# Autodesk Inventor assembly: BrainBoxV1
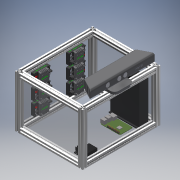
[picture p0: Inventor's stored thumbnail of the model, 180x180]
Saved by Autodesk Inventor 2018 (Build 220112000, 112)
## iProperties
Created: 2019-01-09
Part Number: BrainBoxV1
Document SubType Name: Assembly
Designer: snipe
Author: snipe
## Documents named in this file (14)
- E:\Clark\Assets\BrainBoxV1.iam
- E:\Clark\Assets\Profile_BaseModel_20mm.ipt
- E:\Clark\Assets\Profile_BaseModel_20mm\Profile_BaseModel_20mm-14.ipt
- E:\Clark\Assets\Profile_BaseModel_20mm\Profile_BaseModel_20mm-12.ipt
- E:\Clark\Assets\Profile_BaseModel_20mm\Profile_BaseModel_20mm-11.ipt
- E:\Clark\Assets\PlexiPart\PlexiPart-01.ipt
- E:\Clark\Assets\PlexiPart.ipt
- E:\Clark\Assets\PlexiPart\PlexiPart-02.ipt
- E:\Clark\Assets\PlexiPart\PlexiPart-03.ipt
- E:\Clark\Assets\RPi3Mock.ipt
- E:\Clark\Assets\Netgear Router.ipt
- E:\Clark\Assets\PowerRegulator5V.ipt
- E:\Clark\Assets\Talon.iam
- E:\Clark\Assets\Kinect.iam
## Components (27 placed, 11 different names)
1. Profile_BaseModel_20mm-14:1 — Mate:1, Mate:2, Flush:1, Flush:2, Flush:5, Flush:6, Mate:8, Flush:17, Flush:18, Mate:18, Symmetry:2
2. Profile_BaseModel_20mm-14:2 — Mate:3, Flush:3, Flush:4, Flush:7, Mate:22, Mate:24
3. Profile_BaseModel_20mm-12:5 — Mate:1, Flush:5, Flush:6, Flush:7, Mate:12, Mate:13, Mate:21, Flush:26
4. Profile_BaseModel_20mm-12:6 — Mate:2, Mate:3, Flush:1, Flush:2, Flush:3, Flush:4
5. Profile_BaseModel_20mm-14:7 — Mate:7, Flush:15, Flush:16, Mate:9, Flush:19, Flush:20, Mate:19, Symmetry:2
6. Profile_BaseModel_20mm-14:8 — Mate:10, Flush:21, Flush:22, Mate:11, Flush:23, Flush:24
7. Profile_BaseModel_20mm-12:9 — Mate:20, Mate:27
8. Profile_BaseModel_20mm-12:10 — Mate:50
9. Profile_BaseModel_20mm-11:11 — Mate:7, Flush:15, Flush:16, Mate:8, Flush:17, Flush:18, Mate:48
10. Profile_BaseModel_20mm-11:12 — Mate:9, Flush:19, Flush:20, Mate:14, Mate:17, Mate:26
11. Profile_BaseModel_20mm-11:13 — Mate:10, Flush:21, Flush:22, Mate:51, Mate:55, Flush:37
12. Profile_BaseModel_20mm-11:14 — Mate:11, Flush:23, Flush:24, Mate:23, Mate:25, Mate:54
13. PlexiPart-01:1 — Mate:12, Mate:13, Mate:14, Mate:34, Mate:49, Mate:53
14. PlexiPart-02:3 — Mate:19, Mate:20, Mate:27
15. PlexiPart-02:4 — Mate:21, Mate:22, Flush:26
16. PlexiPart-03:5 — Mate:23, Mate:24, Mate:25
17. PlexiPart-03:6 — Mate:17, Mate:18, Mate:26, Mate:41, Mate:42, Mate:43, Mate:44, Mate:45, Mate:46
18. Talon:7 [sub-assembly] — Mate:41, Flush:28, Flush:31, Mate:47, Symmetry:1
19. Talon:8 [sub-assembly] — Mate:42, Flush:27, Flush:28, Flush:32
20. Talon:9 [sub-assembly] — Mate:43, Flush:27, Flush:33
21. Talon:10 [sub-assembly] — Mate:44, Flush:29, Flush:31, Mate:47, Symmetry:1, Flush:35, Mate:48
22. Talon:11 [sub-assembly] — Mate:45, Flush:29, Flush:30, Flush:32, Flush:35, Flush:36
23. Talon:12 [sub-assembly] — Mate:46, Flush:30, Flush:33, Flush:36
24. RPi3Mock:1 — Mate:34, Mate:52
25. Netgear Router:1 — Mate:49, Mate:50, Mate:51, Mate:52
26. PowerRegulator5V:1 — Mate:53, Mate:54
27. Kinect:1 [sub-assembly] — Mate:55, Flush:37
## Relationships (82: Mate 44, Flush 36, Symmetry 2)
- Mate:1: Profile_BaseModel_20mm-14:1 ↔ Profile_BaseModel_20mm-12:5
- Mate:2: Profile_BaseModel_20mm-14:1 ↔ Profile_BaseModel_20mm-12:6
- Mate:3: Profile_BaseModel_20mm-14:2 ↔ Profile_BaseModel_20mm-12:6
- Flush:1: Profile_BaseModel_20mm-14:1 ↔ Profile_BaseModel_20mm-12:6
- Flush:2: Profile_BaseModel_20mm-14:1 ↔ Profile_BaseModel_20mm-12:6
- Flush:3: Profile_BaseModel_20mm-14:2 ↔ Profile_BaseModel_20mm-12:6
- Flush:4: Profile_BaseModel_20mm-14:2 ↔ Profile_BaseModel_20mm-12:6
- Flush:5: Profile_BaseModel_20mm-14:1 ↔ Profile_BaseModel_20mm-12:5
- Flush:6: Profile_BaseModel_20mm-14:1 ↔ Profile_BaseModel_20mm-12:5
- Flush:7: Profile_BaseModel_20mm-14:2 ↔ Profile_BaseModel_20mm-12:5
- [Mate]: Profile_BaseModel_20mm-14:7 ↔ Profile_BaseModel_20mm-12:9
- [Mate]: Profile_BaseModel_20mm-14:7 ↔ Profile_BaseModel_20mm-12:10
- [Mate]: Profile_BaseModel_20mm-14:8 ↔ Profile_BaseModel_20mm-12:10
- [Flush]: Profile_BaseModel_20mm-14:7 ↔ Profile_BaseModel_20mm-12:10
- [Flush]: Profile_BaseModel_20mm-14:7 ↔ Profile_BaseModel_20mm-12:10
- [Flush]: Profile_BaseModel_20mm-14:8 ↔ Profile_BaseModel_20mm-12:10
- [Flush]: Profile_BaseModel_20mm-14:8 ↔ Profile_BaseModel_20mm-12:10
- [Flush]: Profile_BaseModel_20mm-14:7 ↔ Profile_BaseModel_20mm-12:9
- [Flush]: Profile_BaseModel_20mm-14:7 ↔ Profile_BaseModel_20mm-12:9
- [Flush]: Profile_BaseModel_20mm-14:8 ↔ Profile_BaseModel_20mm-12:9
- Mate:7: Profile_BaseModel_20mm-14:7 ↔ Profile_BaseModel_20mm-11:11
- Flush:15: Profile_BaseModel_20mm-14:7 ↔ Profile_BaseModel_20mm-11:11
- Flush:16: Profile_BaseModel_20mm-14:7 ↔ Profile_BaseModel_20mm-11:11
- Mate:8: Profile_BaseModel_20mm-14:1 ↔ Profile_BaseModel_20mm-11:11
- Flush:17: Profile_BaseModel_20mm-14:1 ↔ Profile_BaseModel_20mm-11:11
- Flush:18: Profile_BaseModel_20mm-14:1 ↔ Profile_BaseModel_20mm-11:11
- Mate:9: Profile_BaseModel_20mm-14:7 ↔ Profile_BaseModel_20mm-11:12
- Flush:19: Profile_BaseModel_20mm-14:7 ↔ Profile_BaseModel_20mm-11:12
- Flush:20: Profile_BaseModel_20mm-14:7 ↔ Profile_BaseModel_20mm-11:12
- Mate:10: Profile_BaseModel_20mm-14:8 ↔ Profile_BaseModel_20mm-11:13
- Flush:21: Profile_BaseModel_20mm-14:8 ↔ Profile_BaseModel_20mm-11:13
- Flush:22: Profile_BaseModel_20mm-14:8 ↔ Profile_BaseModel_20mm-11:13
- Mate:11: Profile_BaseModel_20mm-14:8 ↔ Profile_BaseModel_20mm-11:14
- Flush:23: Profile_BaseModel_20mm-14:8 ↔ Profile_BaseModel_20mm-11:14
- Flush:24: Profile_BaseModel_20mm-14:8 ↔ Profile_BaseModel_20mm-11:14
- Mate:12: Profile_BaseModel_20mm-12:5 ↔ PlexiPart-01:1
- Mate:13: Profile_BaseModel_20mm-12:5 ↔ PlexiPart-01:1
- Mate:14: Profile_BaseModel_20mm-11:12 ↔ PlexiPart-01:1
- Mate:17: Profile_BaseModel_20mm-11:12 ↔ PlexiPart-03:6
- Mate:18: Profile_BaseModel_20mm-14:1 ↔ PlexiPart-03:6
- Mate:19: Profile_BaseModel_20mm-14:7 ↔ PlexiPart-02:3
- Mate:20: Profile_BaseModel_20mm-12:9 ↔ PlexiPart-02:3
- Mate:21: Profile_BaseModel_20mm-12:5 ↔ PlexiPart-02:4
- Mate:22: Profile_BaseModel_20mm-14:2 ↔ PlexiPart-02:4
- Mate:23: Profile_BaseModel_20mm-11:14 ↔ PlexiPart-03:5
- Mate:24: Profile_BaseModel_20mm-14:2 ↔ PlexiPart-03:5
- Flush:26: Profile_BaseModel_20mm-12:5 ↔ PlexiPart-02:4
- Mate:25: Profile_BaseModel_20mm-11:14 ↔ PlexiPart-03:5
- Mate:26: Profile_BaseModel_20mm-11:12 ↔ PlexiPart-03:6
- Mate:27: Profile_BaseModel_20mm-12:9 ↔ PlexiPart-02:3
- Mate:34: PlexiPart-01:1 ↔ RPi3Mock:1
- [Mate]: PlexiPart-03:6 ↔ Talon:10
- [Mate]: PlexiPart-03:6 ↔ Talon:11
- [Mate]: PlexiPart-03:6 ↔ Talon:12
- Mate:41: PlexiPart-03:6 ↔ Talon:7
- Mate:42: PlexiPart-03:6 ↔ Talon:8
- Mate:43: PlexiPart-03:6 ↔ Talon:9
- Flush:27: Talon:8 ↔ Talon:9
- Flush:28: Talon:7 ↔ Talon:8
- Mate:44: PlexiPart-03:6 ↔ Talon:10
- Mate:45: PlexiPart-03:6 ↔ Talon:11
- Mate:46: PlexiPart-03:6 ↔ Talon:12
- Flush:29: Talon:10 ↔ Talon:11
- Flush:30: Talon:11 ↔ Talon:12
- Flush:31: Talon:7 ↔ Talon:10
- Flush:32: Talon:8 ↔ Talon:11
- Flush:33: Talon:9 ↔ Talon:12
- Mate:47 (152.4 mm): Talon:7 ↔ Talon:10
- Symmetry:1: Talon:7 ↔ Talon:10
- Symmetry:2: Profile_BaseModel_20mm-14:1 ↔ Profile_BaseModel_20mm-14:7
- Flush:34
- Flush:35 (57.15 mm): Talon:10 ↔ Talon:11
- Flush:36 (57.15 mm): Talon:11 ↔ Talon:12
- Mate:48 (-50.8 mm): Profile_BaseModel_20mm-11:11 ↔ Talon:10
- Mate:49: PlexiPart-01:1 ↔ Netgear Router:1
- Mate:50 (12.7 mm): Profile_BaseModel_20mm-12:10 ↔ Netgear Router:1
- Mate:51: Profile_BaseModel_20mm-11:13 ↔ Netgear Router:1
- Mate:52 (12.7 mm): RPi3Mock:1 ↔ Netgear Router:1
- Mate:53: PlexiPart-01:1 ↔ PowerRegulator5V:1
- Mate:54: Profile_BaseModel_20mm-11:14 ↔ PowerRegulator5V:1
- Mate:55: Profile_BaseModel_20mm-11:13 ↔ Kinect:1
- Flush:37 (-12.7 mm): Profile_BaseModel_20mm-11:13 ↔ Kinect:1
## Named parameters: d10_d2 = 0 mm, d11_d3 = 0 mm, d12_d4 = 0 mm, d13_d5 = 0 mm, d14_d6 = 0 mm, d15_d7 = 0 mm, d16_d8 = 0 mm, d17_d9 = 0 mm, d18_d0 = 0 mm, d19_d1 = 0 mm
